# Autodesk Inventor assembly: Front Panel
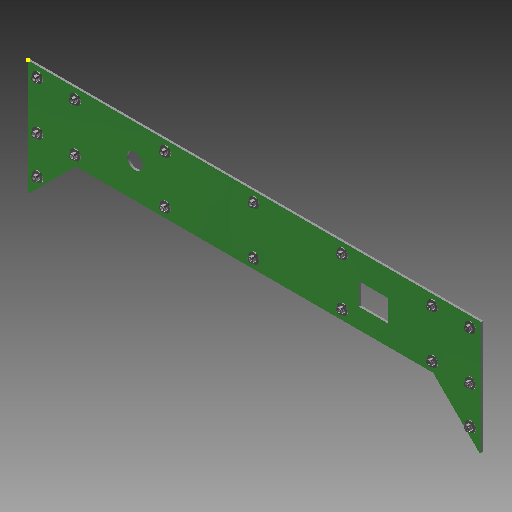
[picture p0: Inventor's stored thumbnail of the model, 512x512]
Saved by Autodesk Inventor 2018 (Build 220112000, 112)
## iProperties
Created: 2016-08-02
Part Number: Front Panel
Document SubType Name: Assembly
Designer: User
Author: User
## Documents named in this file (3)
- C:\Users\Dan\OneDrive\SL-Inventor\The Beast v1.2 PackandGo\Workspaces\Workspace\Front Panel.iam
- C:\Users\Dan\OneDrive\SL-Inventor\The Beast v1.2 PackandGo\Workspaces\Workspace\Acrylic Front Panel - No Graphics.ipt
- C:\Users\Dan\OneDrive\SL-Inventor\The Beast v1.2 PackandGo\Workspaces\Workspace\BoltandTee.iam
## Components (17 placed, 2 different names)
1. Acrylic Front Panel - No Graphics:1
2. BoltandTee:1 [sub-assembly]
3. BoltandTee:2 [sub-assembly]
4. BoltandTee:3 [sub-assembly]
5. BoltandTee:4 [sub-assembly]
6. BoltandTee:5 [sub-assembly]
7. BoltandTee:6 [sub-assembly]
8. BoltandTee:7 [sub-assembly]
9. BoltandTee:8 [sub-assembly]
10. BoltandTee:9 [sub-assembly]
11. BoltandTee:10 [sub-assembly]
12. BoltandTee:11 [sub-assembly]
13. BoltandTee:12 [sub-assembly]
14. BoltandTee:13 [sub-assembly]
15. BoltandTee:14 [sub-assembly]
16. BoltandTee:15 [sub-assembly]
17. BoltandTee:16 [sub-assembly]
## Relationships (16: Mate 14, Insert 2)
- [Mate]: Acrylic Front Panel - No Graphics:1 ↔ BoltandTee:1
- [Mate]: Acrylic Front Panel - No Graphics:1 ↔ BoltandTee:2
- [Mate]: Acrylic Front Panel - No Graphics:1 ↔ BoltandTee:3
- [Mate]: Acrylic Front Panel - No Graphics:1 ↔ BoltandTee:4
- [Mate]: Acrylic Front Panel - No Graphics:1 ↔ BoltandTee:5
- [Mate]: Acrylic Front Panel - No Graphics:1 ↔ BoltandTee:6
- [Mate]: Acrylic Front Panel - No Graphics:1 ↔ BoltandTee:7
- [Mate]: Acrylic Front Panel - No Graphics:1 ↔ BoltandTee:9
- [Mate]: Acrylic Front Panel - No Graphics:1 ↔ BoltandTee:8
- [Mate]: Acrylic Front Panel - No Graphics:1 ↔ BoltandTee:12
- [Mate]: Acrylic Front Panel - No Graphics:1 ↔ BoltandTee:13
- [Mate]: Acrylic Front Panel - No Graphics:1 ↔ BoltandTee:15
- [Mate]: Acrylic Front Panel - No Graphics:1 ↔ BoltandTee:14
- [Mate]: Acrylic Front Panel - No Graphics:1 ↔ BoltandTee:16
- [Insert]: Acrylic Front Panel - No Graphics:1 ↔ BoltandTee:10
- [Insert]: Acrylic Front Panel - No Graphics:1 ↔ BoltandTee:11
